# Autodesk Inventor assembly: a
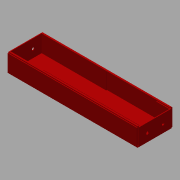
[picture p0: Inventor's stored thumbnail of the model, 180x180]
Saved by Autodesk Inventor 2016 (Build 200138000, 138)
## iProperties
Created: 2015-10-11
Part Number: a
Document SubType Name: Assembly
Designer: daniel
Author: daniel
## Documents named in this file (9)
- C:\Users\daniel\Documents\GitHub\cardboard-stage-metric\stage\a.iam
- C:\Users\daniel\Documents\GitHub\cardboard-stage-metric\stage\aa.ipt
- C:\Users\daniel\Documents\GitHub\cardboard-stage-metric\stage\ab.ipt
- C:\Users\daniel\Documents\GitHub\cardboard-stage-metric\stage\ac.ipt
- C:\Users\daniel\Documents\GitHub\cardboard-stage-metric\stage\ad.ipt
- C:\Users\daniel\Documents\GitHub\cardboard-stage-metric\stage\ae.ipt
- C:\Users\daniel\Documents\GitHub\cardboard-stage-metric\stage\af.ipt
- C:\Users\daniel\Documents\GitHub\cardboard-stage-metric\stage\ah.ipt
- C:\Users\daniel\Documents\GitHub\cardboard-stage-metric\stage\ai.ipt
## Components (13 placed, 8 different names)
1. aa:1 — Mate:1, Mate:2, Mate:3, Mate:4, Mate:5, Mate:6, Flush:1, Flush:2, Mate:7, Mate:8, Flush:4
2. ab:1 — Mate:1, Mate:2, Flush:10
3. ac:1 — Mate:3, Mate:4, Mate:12, Mate:13, Mate:14, Flush:8, Flush:9, Flush:10
4. ad:1 — Mate:5, Mate:6, Flush:1, Mate:9, Mate:10, Mate:15
5. ae:1 — Flush:3, Mate:9, Mate:10, Flush:4, Flush:5, Mate:19, Flush:17
6. af:1 — Mate:16, Flush:11, Flush:12, Flush:16, Mate:19, Flush:17
7. ah:1 — Mate:16, Flush:11, Flush:12
8. ad:2 — Flush:2, Mate:7, Mate:8, Mate:11, Flush:7
9. ae:2 — Flush:3, Flush:5, Mate:11, Mate:18, Mate:20, Flush:18
10. ai:1 — Flush:6, Flush:7, Mate:12, Flush:9
11. ai:2 — Flush:6, Mate:13, Mate:14, Flush:8, Mate:15
12. af:2 — Flush:16, Mate:18, Mate:20, Flush:18
13. ah:2
## Relationships (37: Mate 20, Flush 17)
- Mate:1: aa:1 ↔ ab:1
- Mate:2: aa:1 ↔ ab:1
- Mate:3: aa:1 ↔ ac:1
- Mate:4: aa:1 ↔ ac:1
- Mate:5: aa:1 ↔ ad:1
- Mate:6: aa:1 ↔ ad:1
- Flush:1: aa:1 ↔ ad:1
- Flush:2: aa:1 ↔ ad:2
- Mate:7: aa:1 ↔ ad:2
- Mate:8: aa:1 ↔ ad:2
- Flush:3: ae:1 ↔ ae:2
- Mate:9: ad:1 ↔ ae:1
- Mate:10: ad:1 ↔ ae:1
- Flush:4: aa:1 ↔ ae:1
- Flush:5: ae:1 ↔ ae:2
- Mate:11: ad:2 ↔ ae:2
- Flush:6: ai:1 ↔ ai:2
- Flush:7: ad:2 ↔ ai:1
- Mate:12: ac:1 ↔ ai:1
- Mate:13: ac:1 ↔ ai:2
- Mate:14: ac:1 ↔ ai:2
- Flush:8: ac:1 ↔ ai:2
- Flush:9: ac:1 ↔ ai:1
- Mate:15: ad:1 ↔ ai:2
- Flush:10: ab:1 ↔ ac:1
- Mate:16: af:1 ↔ ah:1
- Flush:11: af:1 ↔ ah:1
- Flush:12: af:1 ↔ ah:1
- [Mate]: af:2 ↔ ah:2
- [Flush]: af:2 ↔ ah:2
- [Flush]: af:2 ↔ ah:2
- Flush:16: af:1 ↔ af:2
- Mate:18: ae:2 ↔ af:2
- Mate:19: ae:1 ↔ af:1
- Flush:17: ae:1 ↔ af:1
- Mate:20: ae:2 ↔ af:2
- Flush:18: ae:2 ↔ af:2
## Named parameters: d28_d25 = 0 mm, d29_d26 = 0 mm, d30_d27 = 0 mm
